# Autodesk Inventor assembly: LIA0005-IO SHIELD ASSY
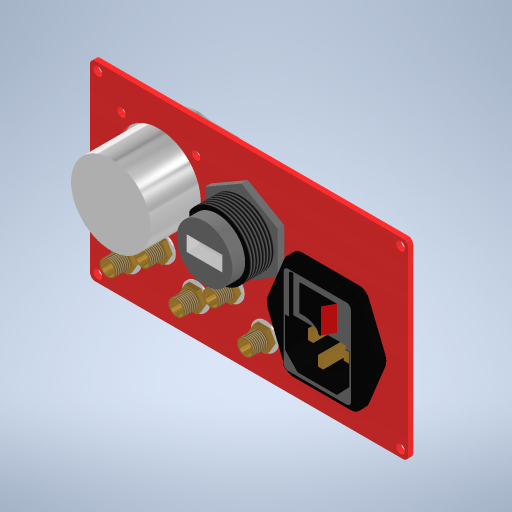
[picture p0: Inventor's stored thumbnail of the model, 512x512]
Saved by Autodesk Inventor 2023 (Build 270158000, 158)
## iProperties
Created: 2023-04-24
Part Number: LIA0005-IO SHIELD ASSY
Document SubType Name: Assembly
Designer: Louis
Author: Louis
## Documents named in this file (9)
- D:\Louis\Documents\Inventor\Interferometry\LIA0005-IO SHIELD ASSY.iam
- D:\Louis\Documents\Inventor\Interferometry\LI0011-IO SHIELD.ipt
- D:\Louis\Documents\Inventor\Interferometry\RS PRO USB 2.0 Cable, Female USB A to Male USB A USB Extension Cable, 200mm.ipt
- D:\Louis\Documents\Inventor\Interferometry\USB NUT.ipt
- D:\Louis\Documents\Inventor\Interferometry\W9011M COAXIAL CONNECTOR.ipt
- D:\Louis\Documents\Inventor\Interferometry\W9011M COAXIAL CONNECTOR WASHER.ipt
- D:\Louis\Documents\Inventor\Interferometry\W9011M COAXIAL CONNECTOR NUT.ipt
- D:\Louis\Documents\Inventor\Interferometry\c-1-1609112-4-c-3d.ipt
- D:\Louis\Documents\Inventor\Interferometry\RJFTV21 X Amphenol Connector.ipt
## Components (20 placed, 8 different names)
1. LI0011-IO SHIELD:1 — Insert:2, Mate:2, Insert:3, Insert:6, Mate:9, Mate:10, Mate:11, Mate:12, Mate:15, Insert:11, Mate:16, Angle:3, Angle:6, Angle:7, Angle:10, Angle:12, Angle:14, Insert:12, Insert:13, Insert:14, Mate:20, Mate:21, Mate:22, Angle:15, Angle:16, Angle:17, Angle:18, Angle:19, Angle:20, Insert:18, Insert:19, Insert:20, Insert:21
2. RS PRO USB 2.0 Cable, Female USB A to Male USB A USB Extension Cable, 200mm:1 — Insert:2, Mate:1, Angle:12
3. USB NUT:1 — Mate:1, Mate:2, Angle:14
4. W9011M COAXIAL CONNECTOR:1 — Insert:3, Mate:5, Angle:7
5. W9011M COAXIAL CONNECTOR:4 — Insert:6, Mate:8, Angle:10
6. W9011M COAXIAL CONNECTOR WASHER:3 — Mate:8, Mate:15, Insert:10
7. W9011M COAXIAL CONNECTOR WASHER:4 — Mate:5, Mate:12, Insert:7
8. W9011M COAXIAL CONNECTOR NUT:1 — Insert:7, Angle:3
9. W9011M COAXIAL CONNECTOR NUT:4 — Insert:10, Angle:6
10. c-1-1609112-4-c-3d:1 — Insert:11, Mate:16
11. W9011M COAXIAL CONNECTOR:5 — Insert:12, Mate:18, Angle:18
12. W9011M COAXIAL CONNECTOR:6 — Insert:13, Mate:17, Angle:19
13. W9011M COAXIAL CONNECTOR:7 — Insert:14, Mate:19, Angle:20
14. W9011M COAXIAL CONNECTOR WASHER:5 — Mate:18, Mate:21, Insert:15
15. W9011M COAXIAL CONNECTOR WASHER:6 — Mate:17, Mate:20, Insert:16
16. W9011M COAXIAL CONNECTOR WASHER:7 — Mate:19, Mate:22, Insert:17
17. W9011M COAXIAL CONNECTOR NUT:5 — Insert:16, Angle:16
18. W9011M COAXIAL CONNECTOR NUT:6 — Insert:15, Angle:15
19. W9011M COAXIAL CONNECTOR NUT:7 — Insert:17, Angle:17
20. RJFTV21 X Amphenol Connector:1 — Insert:18, Insert:19, Insert:20, Insert:21
## Relationships (44: Insert 16, Mate 16, Angle 12)
- Insert:2: LI0011-IO SHIELD:1 ↔ RS PRO USB 2.0 Cable, Female USB A to Male USB A USB Extension Cable, 200mm:1
- Mate:1: RS PRO USB 2.0 Cable, Female USB A to Male USB A USB Extension Cable, 200mm:1 ↔ USB NUT:1
- Mate:2: LI0011-IO SHIELD:1 ↔ USB NUT:1
- Insert:3: LI0011-IO SHIELD:1 ↔ W9011M COAXIAL CONNECTOR:1
- Insert:6: LI0011-IO SHIELD:1 ↔ W9011M COAXIAL CONNECTOR:4
- Mate:5: W9011M COAXIAL CONNECTOR:1 ↔ W9011M COAXIAL CONNECTOR WASHER:4
- Mate:8: W9011M COAXIAL CONNECTOR:4 ↔ W9011M COAXIAL CONNECTOR WASHER:3
- Mate:9: LI0011-IO SHIELD:1
- Mate:10: LI0011-IO SHIELD:1
- Mate:11: LI0011-IO SHIELD:1
- Mate:12: LI0011-IO SHIELD:1 ↔ W9011M COAXIAL CONNECTOR WASHER:4
- Mate:15: LI0011-IO SHIELD:1 ↔ W9011M COAXIAL CONNECTOR WASHER:3
- Insert:7: W9011M COAXIAL CONNECTOR WASHER:4 ↔ W9011M COAXIAL CONNECTOR NUT:1
- Insert:10: W9011M COAXIAL CONNECTOR WASHER:3 ↔ W9011M COAXIAL CONNECTOR NUT:4
- Insert:11: LI0011-IO SHIELD:1 ↔ c-1-1609112-4-c-3d:1
- Mate:16: LI0011-IO SHIELD:1 ↔ c-1-1609112-4-c-3d:1
- Angle:3 (0 deg): LI0011-IO SHIELD:1 ↔ W9011M COAXIAL CONNECTOR NUT:1
- Angle:6 (0 deg): LI0011-IO SHIELD:1 ↔ W9011M COAXIAL CONNECTOR NUT:4
- Angle:7 (0 deg): LI0011-IO SHIELD:1 ↔ W9011M COAXIAL CONNECTOR:1
- Angle:10 (0 deg): LI0011-IO SHIELD:1 ↔ W9011M COAXIAL CONNECTOR:4
- Angle:12 (0 deg): LI0011-IO SHIELD:1 ↔ RS PRO USB 2.0 Cable, Female USB A to Male USB A USB Extension Cable, 200mm:1
- Angle:14 (0 deg): LI0011-IO SHIELD:1 ↔ USB NUT:1
- Insert:12: LI0011-IO SHIELD:1 ↔ W9011M COAXIAL CONNECTOR:5
- Insert:13: LI0011-IO SHIELD:1 ↔ W9011M COAXIAL CONNECTOR:6
- Insert:14: LI0011-IO SHIELD:1 ↔ W9011M COAXIAL CONNECTOR:7
- Mate:17: W9011M COAXIAL CONNECTOR:6 ↔ W9011M COAXIAL CONNECTOR WASHER:6
- Mate:18: W9011M COAXIAL CONNECTOR:5 ↔ W9011M COAXIAL CONNECTOR WASHER:5
- Mate:19: W9011M COAXIAL CONNECTOR:7 ↔ W9011M COAXIAL CONNECTOR WASHER:7
- Mate:20: LI0011-IO SHIELD:1 ↔ W9011M COAXIAL CONNECTOR WASHER:6
- Mate:21: LI0011-IO SHIELD:1 ↔ W9011M COAXIAL CONNECTOR WASHER:5
- Mate:22: LI0011-IO SHIELD:1 ↔ W9011M COAXIAL CONNECTOR WASHER:7
- Insert:15: W9011M COAXIAL CONNECTOR WASHER:5 ↔ W9011M COAXIAL CONNECTOR NUT:6
- Insert:16: W9011M COAXIAL CONNECTOR WASHER:6 ↔ W9011M COAXIAL CONNECTOR NUT:5
- Insert:17: W9011M COAXIAL CONNECTOR WASHER:7 ↔ W9011M COAXIAL CONNECTOR NUT:7
- Angle:15 (0 deg): LI0011-IO SHIELD:1 ↔ W9011M COAXIAL CONNECTOR NUT:6
- Angle:16 (0 deg): LI0011-IO SHIELD:1 ↔ W9011M COAXIAL CONNECTOR NUT:5
- Angle:17 (0 deg): LI0011-IO SHIELD:1 ↔ W9011M COAXIAL CONNECTOR NUT:7
- Angle:18 (0 deg): LI0011-IO SHIELD:1 ↔ W9011M COAXIAL CONNECTOR:5
- Angle:19 (0 deg): LI0011-IO SHIELD:1 ↔ W9011M COAXIAL CONNECTOR:6
- Angle:20 (0 deg): LI0011-IO SHIELD:1 ↔ W9011M COAXIAL CONNECTOR:7
- Insert:18: LI0011-IO SHIELD:1 ↔ RJFTV21 X Amphenol Connector:1
- Insert:19: LI0011-IO SHIELD:1 ↔ RJFTV21 X Amphenol Connector:1
- Insert:20: LI0011-IO SHIELD:1 ↔ RJFTV21 X Amphenol Connector:1
- Insert:21: LI0011-IO SHIELD:1 ↔ RJFTV21 X Amphenol Connector:1
